# Autodesk Inventor assembly: CANcoder Assembly
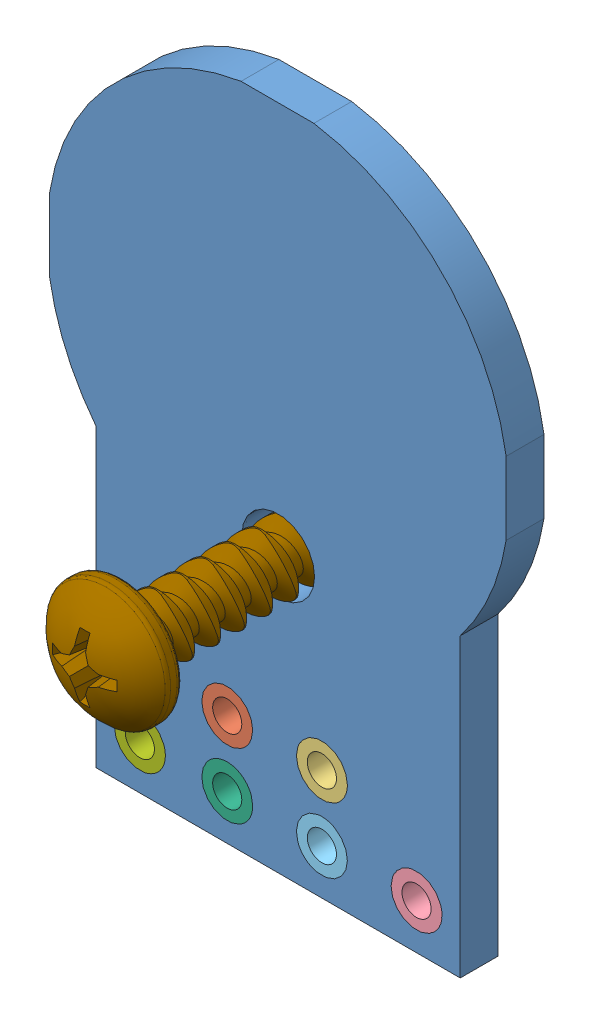
[picture p0: shaded view drawn from the part files that the assembly names]
Saved by Autodesk Inventor 2023 (Build 270158000, 158)
## iProperties
Created: 2023-03-28
Part Number: CANcoder Assembly
Document SubType Name: Assembly
Designer: jackc
Author: jackc
## Documents named in this file (10)
- G:\.shortcut-targets-by-id\1MkDWIt6nIPqRnJSGLfoCUaNz0aFopGUn\1939_Arnold\2_Design\2023-2024\Parts\Swerve\CANcoder Assembly.iam
- G:\.shortcut-targets-by-id\1MkDWIt6nIPqRnJSGLfoCUaNz0aFopGUn\1939_Arnold\2_Design\2023-2024\Parts\Swerve\CANcoder PCA.ipt
- G:\.shortcut-targets-by-id\1MkDWIt6nIPqRnJSGLfoCUaNz0aFopGUn\1939_Arnold\2_Design\2023-2024\Parts\Swerve\CANcoder PCA_1.ipt
- G:\.shortcut-targets-by-id\1MkDWIt6nIPqRnJSGLfoCUaNz0aFopGUn\1939_Arnold\2_Design\2023-2024\Parts\Swerve\CANcoder PCA_2.ipt
- G:\.shortcut-targets-by-id\1MkDWIt6nIPqRnJSGLfoCUaNz0aFopGUn\1939_Arnold\2_Design\2023-2024\Parts\Swerve\CANcoder PCA_3.ipt
- G:\.shortcut-targets-by-id\1MkDWIt6nIPqRnJSGLfoCUaNz0aFopGUn\1939_Arnold\2_Design\2023-2024\Parts\Swerve\CANcoder PCA_4.ipt
- G:\.shortcut-targets-by-id\1MkDWIt6nIPqRnJSGLfoCUaNz0aFopGUn\1939_Arnold\2_Design\2023-2024\Parts\Swerve\CANcoder PCA_5.ipt
- G:\.shortcut-targets-by-id\1MkDWIt6nIPqRnJSGLfoCUaNz0aFopGUn\1939_Arnold\2_Design\2023-2024\Parts\Swerve\CANcoder PCA_6.ipt
- G:\.shortcut-targets-by-id\1MkDWIt6nIPqRnJSGLfoCUaNz0aFopGUn\1939_Arnold\2_Design\2023-2024\Parts\Swerve\CANcoder PCA_7.ipt
- G:\.shortcut-targets-by-id\1MkDWIt6nIPqRnJSGLfoCUaNz0aFopGUn\1939_Arnold\2_Design\2023-2024\Parts\Swerve\CANcoder Screw.ipt
## Components (9 placed, 9 different names)
1. CANcoder PCA — Mate:1, Flush:1, Mate:2, Flush:2, Mate:3, Flush:3, Mate:4, Flush:4, Mate:5, Flush:5, Mate:6, Flush:6, Mate:7, Flush:7, Flush:8, Mate:8
2. CANcoder PCA_1 — Mate:2, Flush:2
3. CANcoder PCA_2 — Mate:4, Flush:4
4. CANcoder PCA_3 — Mate:6, Flush:6
5. CANcoder PCA_4 — Mate:5, Flush:5
6. CANcoder PCA_5 — Mate:3, Flush:3
7. CANcoder PCA_6 — Mate:1, Flush:1
8. CANcoder PCA_7 — Mate:7, Flush:7, Flush:8
9. CANcoder Screw — Mate:8
## Relationships (16: Mate 8, Flush 8)
- Mate:1: CANcoder PCA ↔ CANcoder PCA_6
- Flush:1: CANcoder PCA ↔ CANcoder PCA_6
- Mate:2: CANcoder PCA ↔ CANcoder PCA_1
- Flush:2: CANcoder PCA ↔ CANcoder PCA_1
- Mate:3: CANcoder PCA ↔ CANcoder PCA_5
- Flush:3: CANcoder PCA ↔ CANcoder PCA_5
- Mate:4: CANcoder PCA ↔ CANcoder PCA_2
- Flush:4: CANcoder PCA ↔ CANcoder PCA_2
- Mate:5: CANcoder PCA ↔ CANcoder PCA_4
- Flush:5: CANcoder PCA ↔ CANcoder PCA_4
- Mate:6: CANcoder PCA ↔ CANcoder PCA_3
- Flush:6: CANcoder PCA ↔ CANcoder PCA_3
- Mate:7 (0.127 mm): CANcoder PCA ↔ CANcoder PCA_7
- Flush:7 (12.192 mm): CANcoder PCA ↔ CANcoder PCA_7
- Flush:8 (3.7084 mm): CANcoder PCA ↔ CANcoder PCA_7
- Mate:8: CANcoder PCA ↔ CANcoder Screw
